# Autodesk Inventor assembly: Cathode Assembly
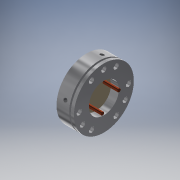
[picture p0: Inventor's stored thumbnail of the model, 180x180]
Saved by Autodesk Inventor 2017.3 (Build 213256000, 256)
## iProperties
Created: 2017-02-08
Part Number: Cathode Assembly
Document SubType Name: Assembly
Designer: Mac
Author: Mac
## Documents named in this file (4)
- C:\Users\Mac\Desktop\UNR Coltrims\eGun Final Design\Cathode\Cathode Assembly.iam
- C:\Users\Mac\Desktop\UNR Coltrims\eGun Final Design\Cathode\Cathode Holder Cap.ipt
- C:\Users\Mac\Desktop\UNR Coltrims\eGun Final Design\Cathode\Cathode Holder.ipt
- C:\Users\Mac\Desktop\UNR Coltrims\eGun Final Design\Cathode\Cathode.ipt
## Components (3 placed, 3 different names)
1. Cathode Holder Cap:1 — Mate:3, Mate:4, Mate:5, Mate:6
2. Cathode Holder:1 — Mate:1, Mate:2, Mate:3, Mate:5
3. Cathode:1 — Mate:1, Mate:2, Mate:4, Mate:6
## Relationships (6: Mate 6)
- Mate:1: Cathode Holder:1 ↔ Cathode:1
- Mate:2: Cathode Holder:1 ↔ Cathode:1
- Mate:3: Cathode Holder Cap:1 ↔ Cathode Holder:1
- Mate:4: Cathode Holder Cap:1 ↔ Cathode:1
- Mate:5: Cathode Holder Cap:1 ↔ Cathode Holder:1
- Mate:6: Cathode Holder Cap:1 ↔ Cathode:1
